# Autodesk Inventor assembly: VPA15AS-6J
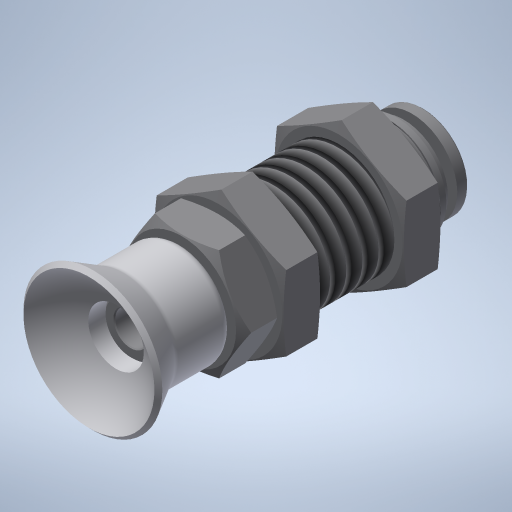
[picture p0: Inventor's stored thumbnail of the model, 512x512]
Saved by Autodesk Inventor 2024.1 (Build 281209000, 209)
## iProperties
Created: 2023-10-05
Part Number: VPA15AS-6J
Catalog Web Link: www.cadenas.de
Description: VPA_R/A-J-Push-in fitting type
Vendor: PISCO_JP
Document SubType Name: Assembly
Designer: psAdmin
Manufacturer: PISCO_JP
Mass: 3.88585 g
Surface Area: 35.4963 cm^2
Volume: 3.88585 cm^3
Density: 1 g/cm^3
Category: PARTsolutions
Company: PISCO_JP
PSOL_IDENT_0: {$CADENAS_DATA/23d-libs/pisco_jp/vacuum_pad_series_r2/vacuum_pad_pad_and_holder_joint_assy/standard_
PSOL_IDENT_1: type/vpa/vpa_ra_j_asmtab.prj},198 {VTYP=3D},{STYP=ASSTAB},{NB=VPA15AS-6J},{LINA=VPA15AS-6J},{NN=VPA_
PSOL_IDENT_2: R/A-J},{DATE=07.10.2020 11:38:11},{GEOMDATE=10.12.2019 10:00:58},{VERSION=},{LINEID=15840},{WBVAR=PM
PSOL_IDENT_3: S,OPECV,OPFH,OPF},{WBNUMERIC=}  {NB=VPA15AS-6J},{LINA=VPA15AS-6J},{KT=DUMMY},{CNSORDERNO=VPA15AS-6J}
PSOL_IDENT_4: ,{PROJECT=Push-in fitting type},{TYPE=VPA},{PTC=A},{PD=15},{ST=},{PJC=6J},{PCC=M4},{PMS=S},{PMSX='N'
PSOL_IDENT_5: ,'N : Nitrile rubber','S','S : Silicone rubber','U','U : Urethane rubber','F','F : Fluoro rubber','N
PSOL_IDENT_6: E','NE : Conductive NBR(Low resistance type)','G','G : NBR Suited for the food sanitation act.','HN'
PSOL_IDENT_7: ,'HN : HNBR','EP','EP : EPDM'},{HA=VPA-M4-6J},{PS=VP15A_-M4},{L1=26.100},{L2=10.000},{L=36.100},{POS=
PSOL_IDENT_8: 0.000},{PPATH=parts/standard_asmtpl.prj},{OPECVX='', 'No', '-ECV', 'ECV : Fall prevention valve'},{O
PSOL_IDENT_9: PECV=},{OPFHX='','No','-FH','FH : Free holder swing angle 30','-FHH','FHH : Free holder swing angle
PSOL_IDENT_10: 15'},{OPFH=},{OPFX='', 'No', '-F15', 'F15 : Filter (Filtration area 1.7 cm^2)'},{OPF=}
NB: VPA15AS-6J
NN: VPA_R/A-J
NT: Push-in fitting type
NBSYN: $CNSORDERNO.
LINA: VPA15AS-6J
CATALOG: NIHON PISCO CO., LTD
CNSORDERNO: VPA15AS-6J
TYPE: VPA
PTC: A
PD: 15
PJC: 6J
PCC: M4
PMS: S : Silicone rubber
OPECV: No
OPFH: No
OPF: No
SUPPLIER: PISCO_JP
ARTICLENO: VPA15AS-6J
BOMINFO: VPA15AS-6J
CREATOR: CADENAS GmbH
Title: VPA15AS-6J
Author: Cadenas PARTsolutions
Comments: Push-in fitting type
## Documents named in this file (5)
- C:\Users\haruy\OneDrive - Kyushu University\cad\000_parts\吸着パッド\pad-15\VPA15AS-6J.iam
- C:\Users\haruy\OneDrive - Kyushu University\cad\000_parts\吸着パッド\pad-15\VP15AS.ipt
- C:\Users\haruy\OneDrive - Kyushu University\cad\000_parts\吸着パッド\pad-15\VPM46-6.ipt
- C:\Users\haruy\OneDrive - Kyushu University\cad\000_parts\吸着パッド\pad-15\FVPA106J.ipt
- C:\Users\haruy\OneDrive - Kyushu University\cad\000_parts\吸着パッド\pad-15\MN12P1(MNF12P1).ipt
## Components (5 placed, 4 different names)
1. VP15AS:1 — IP_screw_XY@1 <-> IP_screw_XY@2, IP_screw_Z@1 <-> IP_screw_Z@2, IP_screw_YZ@1 <-> IP_screw_YZ@2
2. VPM46-6:1 — IP_screw_XY@1 <-> IP_screw_XY@2, IP_screw_Z@1 <-> IP_screw_Z@2, IP_screw_YZ@1 <-> IP_screw_YZ@2
3. FVPA106J:1 — IP_NUT1_XY@3 <-> IP_Holder_XY@4, IP_NUT1_Z@3 <-> IP_Holder_Z@4, IP_NUT1_YZ@3 <-> IP_Holder_YZ@4, IP_NUT2_XY@3 <-> IP_Holder_XY@5, IP_NUT2_Z@3 <-> IP_Holder_Z@5, IP_NUT2_YZ@3 <-> IP_Holder_YZ@5
4. MN12P1(MNF12P1):1 — IP_NUT1_XY@3 <-> IP_Holder_XY@4, IP_NUT1_Z@3 <-> IP_Holder_Z@4, IP_NUT1_YZ@3 <-> IP_Holder_YZ@4
5. MN12P1(MNF12P1):2 — IP_NUT2_XY@3 <-> IP_Holder_XY@5, IP_NUT2_Z@3 <-> IP_Holder_Z@5, IP_NUT2_YZ@3 <-> IP_Holder_YZ@5
## Relationships (9: Mate 5, Angle 3, Flush 1)
- IP_screw_XY@1 <-> IP_screw_XY@2 [Flush]: VP15AS:1 ↔ VPM46-6:1
- IP_screw_Z@1 <-> IP_screw_Z@2 [Mate]: VP15AS:1 ↔ VPM46-6:1
- IP_screw_YZ@1 <-> IP_screw_YZ@2 [Angle] (0 deg): VP15AS:1 ↔ VPM46-6:1
- IP_NUT1_XY@3 <-> IP_Holder_XY@4 [Mate] (-7 mm): FVPA106J:1 ↔ MN12P1(MNF12P1):1
- IP_NUT1_Z@3 <-> IP_Holder_Z@4 [Mate]: FVPA106J:1 ↔ MN12P1(MNF12P1):1
- IP_NUT1_YZ@3 <-> IP_Holder_YZ@4 [Angle] (0 deg): FVPA106J:1 ↔ MN12P1(MNF12P1):1
- IP_NUT2_XY@3 <-> IP_Holder_XY@5 [Mate]: FVPA106J:1 ↔ MN12P1(MNF12P1):2
- IP_NUT2_Z@3 <-> IP_Holder_Z@5 [Mate]: FVPA106J:1 ↔ MN12P1(MNF12P1):2
- IP_NUT2_YZ@3 <-> IP_Holder_YZ@5 [Angle] (0 deg): FVPA106J:1 ↔ MN12P1(MNF12P1):2
